# Autodesk Inventor assembly: FEAandWelding
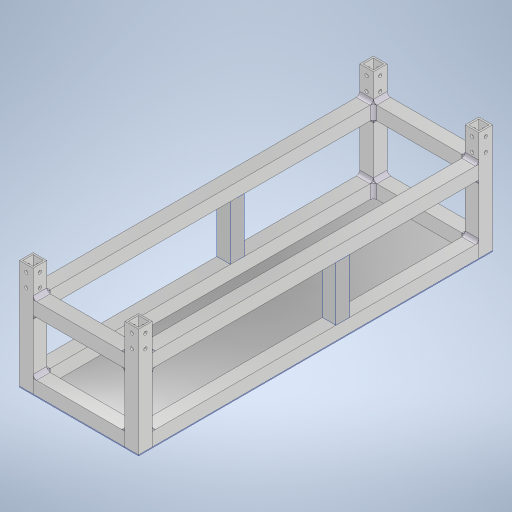
[picture p0: Inventor's stored thumbnail of the model, 512x512]
Saved by Autodesk Inventor 2023 (Build 270158000, 158)
## iProperties
Created: 2022-09-19
Part Number: FEAandWelding
Document SubType Name: Weldment
Designer: seene
Weld Material: Aluminum 6061, Welded
Author: seene
## Documents named in this file (10)
- C:\Users\seene\Desktop\Stony Brook\SBRT\RoboRescue\GrabCAD\Robocup Rescue\Chassis\Frame\FEAandWelding\FEAandWelding.iam
- C:\Users\seene\Desktop\Stony Brook\SBRT\RoboRescue\GrabCAD\Robocup Rescue\Chassis\Frame\Centerpiece\Centerpiece_Frame.iam
- Centerpiece_Frame.iam
- C:\Users\seene\Desktop\Stony Brook\SBRT\RoboRescue\GrabCAD\Robocup Rescue\Chassis\Frame\Centerpiece\Centerpiece_parts\Centerpiece_MiddleSupport.ipt
- C:\Users\seene\Desktop\Stony Brook\SBRT\RoboRescue\GrabCAD\Robocup Rescue\Chassis\Frame\FEAandWelding\FEAandWelding\AIP\FEA\e3ixfb5nk.fins
- C:\Users\seene\Desktop\Stony Brook\SBRT\RoboRescue\GrabCAD\Robocup Rescue\Chassis\Frame\FEAandWelding\FEAandWelding\AIP\FEA\e3ixfb5nk.fsat
- C:\Users\seene\Desktop\Stony Brook\SBRT\RoboRescue\GrabCAD\Robocup Rescue\Chassis\Frame\FEAandWelding\FEAandWelding\AIP\FEA\e3ixfb5nk.ftes
- C:\Users\seene\Desktop\Stony Brook\SBRT\RoboRescue\GrabCAD\Robocup Rescue\Chassis\Frame\FEAandWelding\FEAandWelding\AIP\FEA\e3ixfb5nk.fwiz
- C:\Users\seene\Desktop\Stony Brook\SBRT\RoboRescue\GrabCAD\Robocup Rescue\Chassis\Frame\FEAandWelding\FEAandWelding\AIP\FEA\e3ixfb5vk.fmsh
- C:\Users\seene\Desktop\Stony Brook\SBRT\RoboRescue\GrabCAD\Robocup Rescue\Chassis\Frame\FEAandWelding\FEAandWelding\AIP\FEA\e3ixfb5vl.fres
## Components (3 placed, 2 different names)
1. Centerpiece_Frame:1 [sub-assembly] — Flush:1, Mate:1, Flush:2, Mate:2, Flush:3
2. Centerpiece_MiddleSupport:1 — Flush:1, Mate:1, Mate:4
3. Centerpiece_MiddleSupport:2 — Mate:2, Flush:3, Mate:3
## Relationships (7: Mate 4, Flush 3)
- Flush:1: Centerpiece_Frame:1 ↔ Centerpiece_MiddleSupport:1
- Mate:1: Centerpiece_Frame:1 ↔ Centerpiece_MiddleSupport:1
- Flush:2 (-279.4 mm): Centerpiece_Frame:1
- Mate:2: Centerpiece_Frame:1 ↔ Centerpiece_MiddleSupport:2
- Flush:3: Centerpiece_Frame:1 ↔ Centerpiece_MiddleSupport:2
- Mate:3: Centerpiece_MiddleSupport:2
- Mate:4: Centerpiece_MiddleSupport:1
## Named parameters: sa_0 = 17792.9, sa_1 = 980.999, sa_2 = 2224.11
note: some values were not read from the file. Shown as the stored number, unit unknown: "sa_0", "sa_1", "sa_2".
